# Autodesk Inventor assembly: mini_drone_assembly
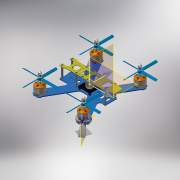
[picture p0: Inventor's stored thumbnail of the model, 180x180]
Saved by Autodesk Inventor 2018 (Build 220112000, 112)
## iProperties
Created: 2018-01-03
Part Number: mini_drone_assembly
Document SubType Name: Assembly
Designer: fbl92568
Author: fbl92568
## Documents named in this file (12)
- C:\Users\FBL92568\Documents\Projects\Mini_Drone\mini_drone_hardware\mini_drone_assembly.iam
- C:\Users\FBL92568\Documents\Projects\Mini_Drone\mini_drone_hardware\components\purchased\base_plate.ipt
- C:\Users\FBL92568\Documents\Projects\Mini_Drone\mini_drone_hardware\components\purchased\frame_spacer.ipt
- C:\Users\FBL92568\Documents\Inventor\Content Center Files\R2018\en-US\ANSI B18.3.4M(1)\ANSI B18.3.4M - M3 x 0.5 x 6(2).ipt
- C:\Users\FBL92568\Documents\Projects\Mini_Drone\mini_drone_hardware\components\purchased\top_plate.ipt
- C:\Users\FBL92568\Documents\Projects\Mini_Drone\mini_drone_hardware\components\purchased\brushless_motor_1000KV.ipt
- C:\Users\FBL92568\Documents\Projects\Mini_Drone\mini_drone_hardware\components\purchased\pdu_riser.ipt
- C:\Users\FBL92568\Documents\Inventor\Content Center Files\R2018\en-US\ANSI B 18.2.4.1 M(1)\ANSI B 18.2.4.1 M - M3 x 0.5Style 1.ipt
- C:\Users\FBL92568\Documents\Projects\Mini_Drone\mini_drone_hardware\components\purchased\matek_systems_pdu.ipt
- C:\Users\FBL92568\Documents\Projects\Mini_Drone\mini_drone_hardware\components\purchased\prop_holder.ipt
- C:\Users\FBL92568\Documents\Projects\Mini_Drone\mini_drone_hardware\components\purchased\40x40x4_prop_blue_cw.ipt
- C:\Users\FBL92568\Documents\Projects\Mini_Drone\mini_drone_hardware\components\designed\landing_foot.ipt
## Components (42 placed, 11 different names)
1. base_plate:1 — Flush:1, Mate:1, Mate:2, Insert:1, Insert:2, Insert:3, Insert:4, Insert:5, Insert:6, Insert:7, Insert:8, Insert:9, Insert:10, Insert:11, Insert:12, Insert:21, Mate:3, Mate:4, Mate:5, Insert:22, Insert:23, Insert:24, Insert:25, Insert:26, Insert:27, Mate:9, Mate:11, Mate:13, Mate:15, Insert:39, Insert:40, Insert:41, Insert:42
2. frame_spacer:1 — Insert:2
3. frame_spacer:2 — Insert:6
4. frame_spacer:3 — Insert:3
5. frame_spacer:4 — Insert:1, Insert:14
6. frame_spacer:5 — Insert:5
7. frame_spacer:6 — Insert:4, Insert:13
8. Broached Hexagon Socket Button Head Cap Screw - Metric M3 x 0.5 x 6:1 — Insert:7
9. Broached Hexagon Socket Button Head Cap Screw - Metric M3 x 0.5 x 6:2 — Insert:8
10. Broached Hexagon Socket Button Head Cap Screw - Metric M3 x 0.5 x 6:3 — Insert:9
11. Broached Hexagon Socket Button Head Cap Screw - Metric M3 x 0.5 x 6:4 — Insert:10
12. Broached Hexagon Socket Button Head Cap Screw - Metric M3 x 0.5 x 6:5 — Insert:11
13. Broached Hexagon Socket Button Head Cap Screw - Metric M3 x 0.5 x 6:6 — Insert:12
14. top_plate:1 — Insert:13, Insert:14, Insert:15, Insert:16, Insert:17, Insert:18, Insert:19, Insert:20
15. Broached Hexagon Socket Button Head Cap Screw - Metric M3 x 0.5 x 6:7 — Insert:15
16. Broached Hexagon Socket Button Head Cap Screw - Metric M3 x 0.5 x 6:8 — Insert:16
17. Broached Hexagon Socket Button Head Cap Screw - Metric M3 x 0.5 x 6:9 — Insert:17
18. Broached Hexagon Socket Button Head Cap Screw - Metric M3 x 0.5 x 6:10 — Insert:18
19. Broached Hexagon Socket Button Head Cap Screw - Metric M3 x 0.5 x 6:11 — Insert:19
20. Broached Hexagon Socket Button Head Cap Screw - Metric M3 x 0.5 x 6:12 — Insert:20
21. brushless_motor_1000KV:1 — Insert:21, Mate:3, Insert:32
22. brushless_motor_1000KV:2 — Mate:4, Mate:5, Insert:34
23. brushless_motor_1000KV:3 — Insert:31, Insert:39, Insert:40
24. brushless_motor_1000KV:4 — Insert:22, Insert:23, Insert:33
25. pdu_riser:1 — Insert:24, Mate:8, Insert:30
26. pdu_riser:2 — Insert:25, Mate:10, Insert:29
27. pdu_riser:3 — Insert:26, Mate:14
28. pdu_riser:4 — Insert:27, Mate:12, Insert:28
29. Hex Nut Metric M3 x 0.5:1 — Mate:8, Mate:9
30. Hex Nut Metric M3 x 0.5:2 — Mate:10, Mate:11
31. Hex Nut Metric M3 x 0.5:3 — Mate:12, Mate:13
32. Hex Nut Metric M3 x 0.5:4 — Mate:14, Mate:15
33. matek_systems_pdu:1 — Insert:28, Insert:29, Insert:30
34. prop_holder:1 — Insert:34, Insert:38
35. prop_holder:2 — Insert:31, Insert:36
36. prop_holder:3 — Insert:33, Insert:37
37. prop_holder:4 — Insert:32, Insert:35
38. 40x40x4_prop_blue_cw:1 — Insert:38
39. 40x40x4_prop_blue_cw:2 — Insert:37
40. 40x40x4_prop_blue_cw:3 — Insert:36
41. 40x40x4_prop_blue_cw:4 — Insert:35
42. landing_foot:1 — Insert:41, Insert:42
## Relationships (56: Insert 42, Mate 13, Flush 1)
- Flush:1: base_plate:1
- Mate:1: base_plate:1
- Mate:2: base_plate:1
- Insert:1: base_plate:1 ↔ frame_spacer:4
- Insert:2: base_plate:1 ↔ frame_spacer:1
- Insert:3: base_plate:1 ↔ frame_spacer:3
- Insert:4: base_plate:1 ↔ frame_spacer:6
- Insert:5: base_plate:1 ↔ frame_spacer:5
- Insert:6: base_plate:1 ↔ frame_spacer:2
- Insert:7: base_plate:1 ↔ Broached Hexagon Socket Button Head Cap Screw - Metric M3 x 0.5 x 6:1
- Insert:8: base_plate:1 ↔ Broached Hexagon Socket Button Head Cap Screw - Metric M3 x 0.5 x 6:2
- Insert:9: base_plate:1 ↔ Broached Hexagon Socket Button Head Cap Screw - Metric M3 x 0.5 x 6:3
- Insert:10: base_plate:1 ↔ Broached Hexagon Socket Button Head Cap Screw - Metric M3 x 0.5 x 6:4
- Insert:11: base_plate:1 ↔ Broached Hexagon Socket Button Head Cap Screw - Metric M3 x 0.5 x 6:5
- Insert:12: base_plate:1 ↔ Broached Hexagon Socket Button Head Cap Screw - Metric M3 x 0.5 x 6:6
- Insert:13: frame_spacer:6 ↔ top_plate:1
- Insert:14: frame_spacer:4 ↔ top_plate:1
- Insert:15: top_plate:1 ↔ Broached Hexagon Socket Button Head Cap Screw - Metric M3 x 0.5 x 6:7
- Insert:16: top_plate:1 ↔ Broached Hexagon Socket Button Head Cap Screw - Metric M3 x 0.5 x 6:8
- Insert:17: top_plate:1 ↔ Broached Hexagon Socket Button Head Cap Screw - Metric M3 x 0.5 x 6:9
- Insert:18: top_plate:1 ↔ Broached Hexagon Socket Button Head Cap Screw - Metric M3 x 0.5 x 6:10
- Insert:19: top_plate:1 ↔ Broached Hexagon Socket Button Head Cap Screw - Metric M3 x 0.5 x 6:11
- Insert:20: top_plate:1 ↔ Broached Hexagon Socket Button Head Cap Screw - Metric M3 x 0.5 x 6:12
- Insert:21: base_plate:1 ↔ brushless_motor_1000KV:1
- Mate:3: base_plate:1 ↔ brushless_motor_1000KV:1
- Mate:4: base_plate:1 ↔ brushless_motor_1000KV:2
- Mate:5: base_plate:1 ↔ brushless_motor_1000KV:2
- Insert:22: base_plate:1 ↔ brushless_motor_1000KV:4
- Insert:23: base_plate:1 ↔ brushless_motor_1000KV:4
- Insert:24: base_plate:1 ↔ pdu_riser:1
- Insert:25: base_plate:1 ↔ pdu_riser:2
- Insert:26: base_plate:1 ↔ pdu_riser:3
- Insert:27: base_plate:1 ↔ pdu_riser:4
- Mate:8: pdu_riser:1 ↔ Hex Nut Metric M3 x 0.5:1
- Mate:9: base_plate:1 ↔ Hex Nut Metric M3 x 0.5:1
- Mate:10: pdu_riser:2 ↔ Hex Nut Metric M3 x 0.5:2
- Mate:11: base_plate:1 ↔ Hex Nut Metric M3 x 0.5:2
- Mate:12: pdu_riser:4 ↔ Hex Nut Metric M3 x 0.5:3
- Mate:13: base_plate:1 ↔ Hex Nut Metric M3 x 0.5:3
- Mate:14: pdu_riser:3 ↔ Hex Nut Metric M3 x 0.5:4
- Mate:15: base_plate:1 ↔ Hex Nut Metric M3 x 0.5:4
- Insert:28: pdu_riser:4 ↔ matek_systems_pdu:1
- Insert:29: pdu_riser:2 ↔ matek_systems_pdu:1
- Insert:30: pdu_riser:1 ↔ matek_systems_pdu:1
- Insert:31: brushless_motor_1000KV:3 ↔ prop_holder:2
- Insert:32: brushless_motor_1000KV:1 ↔ prop_holder:4
- Insert:33: brushless_motor_1000KV:4 ↔ prop_holder:3
- Insert:34: brushless_motor_1000KV:2 ↔ prop_holder:1
- Insert:35: prop_holder:4 ↔ 40x40x4_prop_blue_cw:4
- Insert:36: prop_holder:2 ↔ 40x40x4_prop_blue_cw:3
- Insert:37: prop_holder:3 ↔ 40x40x4_prop_blue_cw:2
- Insert:38: prop_holder:1 ↔ 40x40x4_prop_blue_cw:1
- Insert:39: base_plate:1 ↔ brushless_motor_1000KV:3
- Insert:40: base_plate:1 ↔ brushless_motor_1000KV:3
- Insert:41: base_plate:1 ↔ landing_foot:1
- Insert:42: base_plate:1 ↔ landing_foot:1
